# Autodesk Inventor assembly: the thing
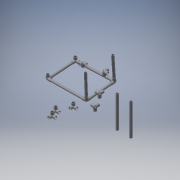
[picture p0: Inventor's stored thumbnail of the model, 180x180]
Saved by Autodesk Inventor 2016 (Build 200138000, 138)
## iProperties
Created: 2017-01-31
Part Number: the thing
Document SubType Name: Assembly
Designer: Student
Author: Student
## Documents named in this file (4)
- C:\Users\Student\Desktop\Noah Code\the thing.iam
- C:\Users\Student\Documents\pvc pipe 1in 1.ipt
- C:\Users\Student\Documents\pvc 1in 3 way elbow.ipt
- C:\Users\Student\Documents\pvc pipe 1in 1ft 1.ipt
## Components (19 placed, 3 different names)
1. pvc pipe 1in 1:1 — Mate:1, Mate:2, Mate:5
2. pvc pipe 1in 1:2 — Mate:9, Mate:10, Mate:12
3. pvc pipe 1in 1:3
4. pvc pipe 1in 1:4
5. pvc 1in 3 way elbow:1
6. pvc 1in 3 way elbow:2
7. pvc 1in 3 way elbow:3 — Mate:1, Mate:2, Mate:3, Mate:4
8. pvc 1in 3 way elbow:4
9. pvc pipe 1in 1ft 1:1 — Mate:3, Mate:4, Mate:11
10. pvc pipe 1in 1ft 1:2 — Mate:6, Mate:7, Mate:8
11. pvc pipe 1in 1ft 1:3 — Mate:13, Mate:14
12. pvc pipe 1in 1ft 1:4 — Mate:15, Mate:16
13. pvc 1in 3 way elbow:5 — Mate:11, Mate:12
14. pvc 1in 3 way elbow:6 — Mate:5, Mate:6, Mate:7, Mate:13, Mate:14
15. pvc 1in 3 way elbow:7 — Mate:8, Mate:9, Mate:10, Mate:15, Mate:16
16. pvc 1in 3 way elbow:8
17. pvc 1in 3 way elbow:9
18. pvc 1in 3 way elbow:10
19. pvc 1in 3 way elbow:11
## Relationships (16: Mate 16)
- Mate:1: pvc pipe 1in 1:1 ↔ pvc 1in 3 way elbow:3
- Mate:2: pvc pipe 1in 1:1 ↔ pvc 1in 3 way elbow:3
- Mate:3: pvc 1in 3 way elbow:3 ↔ pvc pipe 1in 1ft 1:1
- Mate:4: pvc 1in 3 way elbow:3 ↔ pvc pipe 1in 1ft 1:1
- Mate:5: pvc pipe 1in 1:1 ↔ pvc 1in 3 way elbow:6
- Mate:6: pvc pipe 1in 1ft 1:2 ↔ pvc 1in 3 way elbow:6
- Mate:7: pvc pipe 1in 1ft 1:2 ↔ pvc 1in 3 way elbow:6
- Mate:8: pvc pipe 1in 1ft 1:2 ↔ pvc 1in 3 way elbow:7
- Mate:9: pvc pipe 1in 1:2 ↔ pvc 1in 3 way elbow:7
- Mate:10: pvc pipe 1in 1:2 ↔ pvc 1in 3 way elbow:7
- Mate:11: pvc pipe 1in 1ft 1:1 ↔ pvc 1in 3 way elbow:5
- Mate:12: pvc pipe 1in 1:2 ↔ pvc 1in 3 way elbow:5
- Mate:13: pvc pipe 1in 1ft 1:3 ↔ pvc 1in 3 way elbow:6
- Mate:14: pvc pipe 1in 1ft 1:3 ↔ pvc 1in 3 way elbow:6
- Mate:15: pvc pipe 1in 1ft 1:4 ↔ pvc 1in 3 way elbow:7
- Mate:16: pvc pipe 1in 1ft 1:4 ↔ pvc 1in 3 way elbow:7
